# Autodesk Inventor assembly: Tractor_Assembly
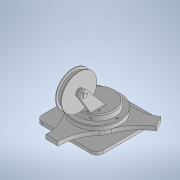
[picture p0: Inventor's stored thumbnail of the model, 180x180]
Saved by Autodesk Inventor 2022 (Build 260153070, 153G)
## iProperties
Created: 2022-03-05
Part Number: Tractor_Assembly
Document SubType Name: Assembly
Designer: a laptop
Author: a laptop
## Documents named in this file (4)
- C:\Users\a laptop\Desktop\MDL_2021_Project\Tractor_Assembly.iam
- C:\Users\a laptop\Desktop\MDL_2021_Project\Tractor_Plates\Tractor_Plates.iam
- C:\Users\a laptop\Desktop\MDL_2021_Project\Return_Spool_Reel\Return_Spool_Mount.iam
- C:\Users\a laptop\Desktop\MDL_2021_Project\AS5600.ipt
## Components (3 placed, 3 different names)
1. Tractor_Plates:1 [sub-assembly] — Mate:1, Mate:2, Mate:4, Mate:5
2. Return_Spool_Mount:1 [sub-assembly] — Mate:1, Mate:2, Mate:6, Mate:7
3. AS5600:1 — Mate:4, Mate:5, Mate:6, Mate:7
## Relationships (6: Mate 6)
- Mate:1: Tractor_Plates:1 ↔ Return_Spool_Mount:1
- Mate:2: Tractor_Plates:1 ↔ Return_Spool_Mount:1
- Mate:4 (5 mm): Tractor_Plates:1 ↔ AS5600:1
- Mate:5: Tractor_Plates:1 ↔ AS5600:1
- Mate:6: Return_Spool_Mount:1 ↔ AS5600:1
- Mate:7: Return_Spool_Mount:1 ↔ AS5600:1
